# Autodesk Inventor assembly: 6wd
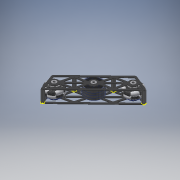
[picture p0: Inventor's stored thumbnail of the model, 180x180]
Saved by Autodesk Inventor 2018.3 (Build 223284000, 284)
## iProperties
Created: 2018-06-26
Part Number: 6wd
Document SubType Name: Assembly
Designer: mzhang
Author: mzhang
## Documents named in this file (8)
- C:\Users\mzhang\3D Objects\6wd.iam
- C:\Users\mzhang\3D Objects\6wdPlate.ipt
- C:\Users\mzhang\Downloads\0_375_Hex_ID_x_1_125_OD_x_0_313_WD_Flanged_Bearing_217-2735.ipt
- C:\Users\mzhang\Downloads\am-2231a+375+Hex+Hub+r3.ipt
- C:\Users\mzhang\Downloads\am-3047_4inDuraOmniV2.ipt
- C:\Users\mzhang\Downloads\am-0234_S25-36LSprocket.ipt
- C:\Users\mzhang\Downloads\am-3435+4IN+Stealth+Wheel+375+HEX+Bore.ipt
- C:\Users\mzhang\3D Objects\6wd rev.ipt
## Components (21 placed, 7 different names)
1. 6wdPlate:1 — Mate:1, Mate:2, Mate:11, Mate:12, Mate:22, Mate:23, Flush:15, Mate:35, Mate:38, Mate:39, Mate:43
2. 0_375_Hex_ID_x_1_125_OD_x_0_313_WD_Flanged_Bearing_217-2735:1 — Mate:1, Mate:2, Flush:8, Flush:9, Mate:6, Mate:26
3. am-2231a+375+Hex+Hub+r3:1 — Mate:3, Mate:4, Mate:5, Flush:8, Flush:9, Mate:6
4. am-3047_4inDuraOmniV2:1 — Mate:3, Mate:4, Mate:5, Mate:25, Tangent:3
5. 0_375_Hex_ID_x_1_125_OD_x_0_313_WD_Flanged_Bearing_217-2735:2 — Mate:11, Mate:12
6. am-2231a+375+Hex+Hub+r3:2
7. am-3047_4inDuraOmniV2:2 — Mate:16, Tangent:1, Mate:34
8. am-0234_S25-36LSprocket:1 — Mate:16, Tangent:1, Flush:14, Mate:33, Mate:34
9. am-0234_S25-36LSprocket:2 — Flush:14, Mate:24, Tangent:2
10. am-3435+4IN+Stealth+Wheel+375+HEX+Bore:1 — Mate:18, Mate:19, Mate:20, Tangent:2
11. am-3435+4IN+Stealth+Wheel+375+HEX+Bore:2 — Mate:18, Mate:19, Mate:20, Flush:12, Mate:21, Flush:13
12. 0_375_Hex_ID_x_1_125_OD_x_0_313_WD_Flanged_Bearing_217-2735:3 — Flush:12, Mate:21, Flush:13, Mate:22, Mate:23, Mate:24
13. am-0234_S25-36LSprocket:3 — Mate:25, Mate:26, Tangent:3
14. 6wdPlate:2 — Flush:15, Mate:35, Mate:36, Mate:37, Mate:40, Mate:41, Mate:42
15. 0_375_Hex_ID_x_1_125_OD_x_0_313_WD_Flanged_Bearing_217-2735:4 — Mate:33
16. 0_375_Hex_ID_x_1_125_OD_x_0_313_WD_Flanged_Bearing_217-2735:5
17. 0_375_Hex_ID_x_1_125_OD_x_0_313_WD_Flanged_Bearing_217-2735:6
18. 6wd rev:1 — Mate:36, Mate:37
19. 6wd rev:2 — Mate:42, Mate:43
20. 6wd rev:3 — Mate:38, Mate:39
21. 6wd rev:4 — Mate:40, Mate:41
## Relationships (50: Mate 39, Flush 8, Tangent 3)
- Mate:1: 6wdPlate:1 ↔ 0_375_Hex_ID_x_1_125_OD_x_0_313_WD_Flanged_Bearing_217-2735:1
- Mate:2: 6wdPlate:1 ↔ 0_375_Hex_ID_x_1_125_OD_x_0_313_WD_Flanged_Bearing_217-2735:1
- Mate:3: am-2231a+375+Hex+Hub+r3:1 ↔ am-3047_4inDuraOmniV2:1
- Mate:4: am-2231a+375+Hex+Hub+r3:1 ↔ am-3047_4inDuraOmniV2:1
- Mate:5: am-2231a+375+Hex+Hub+r3:1 ↔ am-3047_4inDuraOmniV2:1
- Flush:8: 0_375_Hex_ID_x_1_125_OD_x_0_313_WD_Flanged_Bearing_217-2735:1 ↔ am-2231a+375+Hex+Hub+r3:1
- Flush:9: 0_375_Hex_ID_x_1_125_OD_x_0_313_WD_Flanged_Bearing_217-2735:1 ↔ am-2231a+375+Hex+Hub+r3:1
- Mate:6: 0_375_Hex_ID_x_1_125_OD_x_0_313_WD_Flanged_Bearing_217-2735:1 ↔ am-2231a+375+Hex+Hub+r3:1
- [Mate]: am-2231a+375+Hex+Hub+r3:2 ↔ am-3047_4inDuraOmniV2:2
- [Mate]: am-2231a+375+Hex+Hub+r3:2 ↔ am-3047_4inDuraOmniV2:2
- [Mate]: am-2231a+375+Hex+Hub+r3:2 ↔ am-3047_4inDuraOmniV2:2
- [Flush]: 0_375_Hex_ID_x_1_125_OD_x_0_313_WD_Flanged_Bearing_217-2735:2 ↔ am-2231a+375+Hex+Hub+r3:2
- [Flush]: 0_375_Hex_ID_x_1_125_OD_x_0_313_WD_Flanged_Bearing_217-2735:2 ↔ am-2231a+375+Hex+Hub+r3:2
- [Mate]: 0_375_Hex_ID_x_1_125_OD_x_0_313_WD_Flanged_Bearing_217-2735:2 ↔ am-2231a+375+Hex+Hub+r3:2
- Mate:11: 6wdPlate:1 ↔ 0_375_Hex_ID_x_1_125_OD_x_0_313_WD_Flanged_Bearing_217-2735:2
- Mate:12: 6wdPlate:1 ↔ 0_375_Hex_ID_x_1_125_OD_x_0_313_WD_Flanged_Bearing_217-2735:2
- Mate:16: am-3047_4inDuraOmniV2:2 ↔ am-0234_S25-36LSprocket:1
- Tangent:1: am-3047_4inDuraOmniV2:2 ↔ am-0234_S25-36LSprocket:1
- Mate:18: am-3435+4IN+Stealth+Wheel+375+HEX+Bore:1 ↔ am-3435+4IN+Stealth+Wheel+375+HEX+Bore:2
- Mate:19: am-3435+4IN+Stealth+Wheel+375+HEX+Bore:1 ↔ am-3435+4IN+Stealth+Wheel+375+HEX+Bore:2
- Mate:20: am-3435+4IN+Stealth+Wheel+375+HEX+Bore:1 ↔ am-3435+4IN+Stealth+Wheel+375+HEX+Bore:2
- Flush:12: am-3435+4IN+Stealth+Wheel+375+HEX+Bore:2 ↔ 0_375_Hex_ID_x_1_125_OD_x_0_313_WD_Flanged_Bearing_217-2735:3
- Mate:21: am-3435+4IN+Stealth+Wheel+375+HEX+Bore:2 ↔ 0_375_Hex_ID_x_1_125_OD_x_0_313_WD_Flanged_Bearing_217-2735:3
- Flush:13: am-3435+4IN+Stealth+Wheel+375+HEX+Bore:2 ↔ 0_375_Hex_ID_x_1_125_OD_x_0_313_WD_Flanged_Bearing_217-2735:3
- Mate:22: 6wdPlate:1 ↔ 0_375_Hex_ID_x_1_125_OD_x_0_313_WD_Flanged_Bearing_217-2735:3
- Mate:23: 6wdPlate:1 ↔ 0_375_Hex_ID_x_1_125_OD_x_0_313_WD_Flanged_Bearing_217-2735:3
- Flush:14: am-0234_S25-36LSprocket:1 ↔ am-0234_S25-36LSprocket:2
- Mate:24: am-0234_S25-36LSprocket:2 ↔ 0_375_Hex_ID_x_1_125_OD_x_0_313_WD_Flanged_Bearing_217-2735:3
- Tangent:2: am-0234_S25-36LSprocket:2 ↔ am-3435+4IN+Stealth+Wheel+375+HEX+Bore:1
- Mate:25: am-3047_4inDuraOmniV2:1 ↔ am-0234_S25-36LSprocket:3
- Mate:26: 0_375_Hex_ID_x_1_125_OD_x_0_313_WD_Flanged_Bearing_217-2735:1 ↔ am-0234_S25-36LSprocket:3
- Tangent:3: am-3047_4inDuraOmniV2:1 ↔ am-0234_S25-36LSprocket:3
- [Mate]: 6wdPlate:2 ↔ 0_375_Hex_ID_x_1_125_OD_x_0_313_WD_Flanged_Bearing_217-2735:4
- [Mate]: 6wdPlate:2 ↔ 0_375_Hex_ID_x_1_125_OD_x_0_313_WD_Flanged_Bearing_217-2735:4
- [Mate]: 6wdPlate:2 ↔ 0_375_Hex_ID_x_1_125_OD_x_0_313_WD_Flanged_Bearing_217-2735:5
- [Mate]: 6wdPlate:2 ↔ 0_375_Hex_ID_x_1_125_OD_x_0_313_WD_Flanged_Bearing_217-2735:5
- [Mate]: 6wdPlate:2 ↔ 0_375_Hex_ID_x_1_125_OD_x_0_313_WD_Flanged_Bearing_217-2735:6
- [Mate]: 6wdPlate:2 ↔ 0_375_Hex_ID_x_1_125_OD_x_0_313_WD_Flanged_Bearing_217-2735:6
- Mate:33 (6.35 mm): am-0234_S25-36LSprocket:1 ↔ 0_375_Hex_ID_x_1_125_OD_x_0_313_WD_Flanged_Bearing_217-2735:4
- Mate:34: am-3047_4inDuraOmniV2:2 ↔ am-0234_S25-36LSprocket:1
- Flush:15: 6wdPlate:1 ↔ 6wdPlate:2
- Mate:35: 6wdPlate:1 ↔ 6wdPlate:2
- Mate:36: 6wdPlate:2 ↔ 6wd rev:1
- Mate:37: 6wdPlate:2 ↔ 6wd rev:1
- Mate:38: 6wdPlate:1 ↔ 6wd rev:3
- Mate:39: 6wdPlate:1 ↔ 6wd rev:3
- Mate:40: 6wdPlate:2 ↔ 6wd rev:4
- Mate:41: 6wdPlate:2 ↔ 6wd rev:4
- Mate:42: 6wdPlate:2 ↔ 6wd rev:2
- Mate:43: 6wdPlate:1 ↔ 6wd rev:2
## Named parameters: d11_d3 = 0 mm, d12_d4 = 0 mm, d13_d8 = 0 mm, d14_d9 = 0 mm, d15_d10 = 0 mm, d16_d2 = 0 mm, d42_d34 = 0 mm, d43_d35 = 0 mm, d44_d17 = 0 mm, d45_d18 = 0 mm, d46_d0 = 0 mm, d47_d1 = 0 mm
